# Autodesk Inventor assembly: Spider_Robot_Leg_Assembly_V1
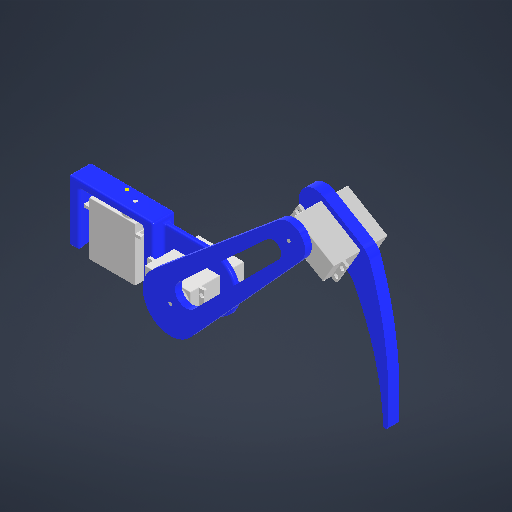
[picture p0: Inventor's stored thumbnail of the model, 512x512]
Saved by Autodesk Inventor 2026.2 (Build 302298010, 298A)
## iProperties
Created: 2026-08-15
Part Number: Spider_Robot_Leg_Assembly_V1
Document SubType Name: Assembly
Designer: Entity
Author: Entity
## Documents named in this file (5)
- C:\Users\Entity\OneDrive\Documents\Bells University of Technology Documents\Autodesk Inventor Projects\Spider_Robot_Leg_Assembly_V1.iam
- C:\Users\Entity\OneDrive\Documents\Bells University of Technology Documents\Autodesk Inventor Projects\Servo Part 1.ipt
- C:\Users\Entity\OneDrive\Documents\Bells University of Technology Documents\Autodesk Inventor Projects\Spider_Robot_Femur_V1.ipt
- C:\Users\Entity\OneDrive\Documents\Bells University of Technology Documents\Autodesk Inventor Projects\Spider_Robot_Tibia_V1.ipt
- C:\Users\Entity\OneDrive\Documents\Bells University of Technology Documents\Autodesk Inventor Projects\Spider_Robot_Coxa_V1.stl
## Components (6 placed, 4 different names)
1. Spider_Robot_Coxa_V1:1 — Rotational:1, Rigid:1
2. Servo Part 1:1 — Rotational:1
3. Servo Part 1:3 — Rigid:1, Rotational:2
4. Spider_Robot_Femur_V1:1 — Rotational:2, Rotational:3
5. Spider_Robot_Tibia_V1:1 — Rigid:2
6. Servo Part 1:5 — Rigid:2, Rotational:3
## Relationships (5: RevoluteJoint 3, WeldJoint 2)
- Rotational:1 [RevoluteJoint]: Spider_Robot_Coxa_V1:1 ↔ Servo Part 1:1
- Rigid:1 [WeldJoint]: Spider_Robot_Coxa_V1:1 ↔ Servo Part 1:3
- Rotational:2 [RevoluteJoint]: Servo Part 1:3 ↔ Spider_Robot_Femur_V1:1
- Rigid:2 [WeldJoint]: Spider_Robot_Tibia_V1:1 ↔ Servo Part 1:5
- Rotational:3 [RevoluteJoint]: Spider_Robot_Femur_V1:1 ↔ Servo Part 1:5
